# Autodesk Inventor assembly: BedAssembly
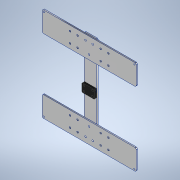
[picture p0: Inventor's stored thumbnail of the model, 180x180]
Saved by Autodesk Inventor 2020.2 (Build 242310000, 310)
## iProperties
Created: 2020-08-19
Part Number: BedAssembly
Document SubType Name: Assembly
Designer: JK
Author: JK
## Documents named in this file (4)
- C:\Users\JK\Documents\Inventor\Anet Upgrade\BedAssembly.iam
- C:\Users\JK\Documents\Inventor\Anet Upgrade\BedCarriageA.ipt
- C:\Users\JK\Documents\Inventor\Anet Upgrade\BedCarriageB.ipt
- C:\Users\JK\Documents\Inventor\Anet Upgrade\Y Belt Attachment A.ipt
## Components (3 placed, 3 different names)
1. BedCarriageA:1 — Mate:1, Mate:2, Flush:1
2. BedCarriageB:1 — Mate:1, Mate:2, Flush:1, Mate:3, Flush:2, Mate:4
3. Y Belt Attachment A:1 — Mate:3, Flush:2, Mate:4
## Relationships (6: Mate 4, Flush 2)
- Mate:1: BedCarriageA:1 ↔ BedCarriageB:1
- Mate:2: BedCarriageA:1 ↔ BedCarriageB:1
- Flush:1: BedCarriageA:1 ↔ BedCarriageB:1
- Mate:3: BedCarriageB:1 ↔ Y Belt Attachment A:1
- Flush:2: BedCarriageB:1 ↔ Y Belt Attachment A:1
- Mate:4: BedCarriageB:1 ↔ Y Belt Attachment A:1
